# Autodesk Inventor assembly: Assembly2
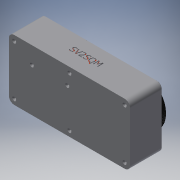
[picture p0: Inventor's stored thumbnail of the model, 180x180]
Saved by Autodesk Inventor 2017.3 (Build 213257000, 257)
## iProperties
Created: 2021-12-05
Part Number: Assembly2
Document SubType Name: Assembly
Designer: TEOS
Author: TEOS
## Documents named in this file (10)
- C:\Users\TEOS\Documents\SDRconsoleMIDIcontroller\Assembly2.iam
- C:\Users\TEOS\Documents\SDRconsoleMIDIcontroller\box.ipt
- C:\Users\TEOS\Documents\SDRconsoleMIDIcontroller\buttons.ipt
- C:\Users\TEOS\Documents\SDRconsoleMIDIcontroller\bottom.ipt
- C:\Users\TEOS\Documents\Inventor\Content Center Files\R2017\en-US\DIN 934\DIN 934 - M27 x 3.ipt
- C:\Users\TEOS\Documents\SDRconsoleMIDIcontroller\arduino_uno.ipt
- C:\Users\TEOS\Documents\SDRconsoleMIDIcontroller\rotary-encoder-knob-69.ipt
- C:\Users\TEOS\Documents\SDRconsoleMIDIcontroller\rotary-encoder-knob-25.ipt
- C:\Users\TEOS\Documents\SDRconsoleMIDIcontroller\rotary-encoder-knob-25_CPY.ipt
- C:\Users\TEOS\Documents\SDRconsoleMIDIcontroller\buttonHolder.ipt
## Components (9 placed, 9 different names)
1. box:1 — Flush:1, Flush:2, Flush:3, Flush:4, Flush:5, Insert:2, Insert:3, Insert:4
2. buttons:1 — Flush:1, Flush:2, Flush:3, Flush:8
3. bottom:1 — Flush:4, Flush:5, Mate:1, Flush:6, Flush:9
4. DIN 934 - replaced by DIN EN 24032/28673/28674 M27:1 — Mate:1
5. arduino_uno:1
6. rotary-encoder-knob-69:1 — Insert:4
7. rotary-encoder-knob-25:1 — Insert:2
8. rotary-encoder-knob-25_CPY:1 — Insert:3
9. buttonHolder:1 — Flush:6, Flush:8, Flush:9
## Relationships (12: Flush 8, Insert 3, Mate 1)
- Flush:1: box:1 ↔ buttons:1
- Flush:2: box:1 ↔ buttons:1
- Flush:3: box:1 ↔ buttons:1
- Flush:4: box:1 ↔ bottom:1
- Flush:5 (-3 mm): box:1 ↔ bottom:1
- Mate:1: bottom:1 ↔ DIN 934 - replaced by DIN EN 24032/28673/28674 M27:1
- Insert:2: box:1 ↔ rotary-encoder-knob-25:1
- Insert:3: box:1 ↔ rotary-encoder-knob-25_CPY:1
- Insert:4: box:1 ↔ rotary-encoder-knob-69:1
- Flush:6: bottom:1 ↔ buttonHolder:1
- Flush:8 (5 mm): buttons:1 ↔ buttonHolder:1
- Flush:9: bottom:1 ↔ buttonHolder:1
